# Autodesk Inventor assembly: plugassembly2
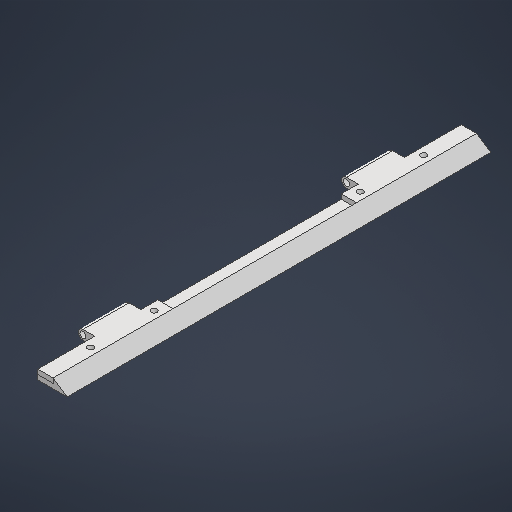
[picture p0: Inventor's stored thumbnail of the model, 512x512]
Saved by Autodesk Inventor 2026.2 (Build 302298010, 298A)
## iProperties
Created: 2026-09-28
Part Number: plugassembly2
Document SubType Name: Assembly
Designer: karol
Author: karol
## Documents named in this file (3)
- C:\Users\karol\OneDrive\Dokumenty\GitHub\bolt_v2\ bolt_v2\CAD\Assemblys\plugassembly2.iam
- C:\Users\karol\OneDrive\Dokumenty\GitHub\bolt_v2\ bolt_v2\CAD\ready parts\plug.ipt
- C:\Users\karol\OneDrive\Dokumenty\GitHub\bolt_v2\ bolt_v2\CAD\ready parts\mocowaniedoplugu.ipt
## Components (2 placed, 2 different names)
1. plug:1 — Flush:1
2. mocowaniedoplugu:1 — Flush:1
## Relationships (1: Flush 1)
- Flush:1: plug:1 ↔ mocowaniedoplugu:1
